# Autodesk Inventor assembly: COTS_ARMA_AR3603_Hinge
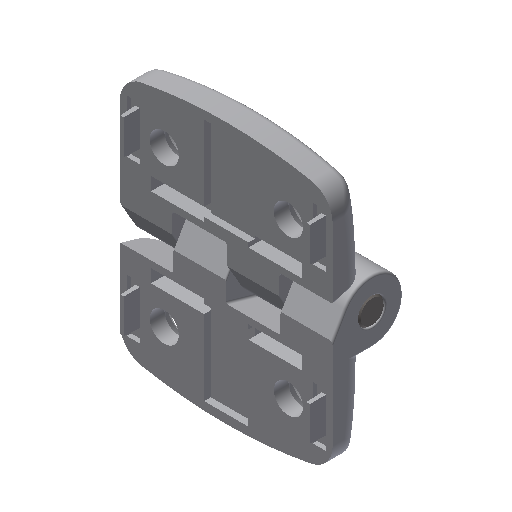
[picture p0: Inventor's stored thumbnail of the model, 512x512]
Saved by Autodesk Inventor 2026.1 (Build 301233000, 233)
## iProperties
Created: 2016-06-24
Part Number: COTS_ARMA_AR3603_Hinge
Material: Ogólny
Document SubType Name: Assembly
Designer: Andrzej
Sending System: Autodesk Inventor 2013
Preprocessor: Autodesk Inventor 2013
Title: \\WIN\Rysunki\Inventor\@System profili aluminiowych\System profili aluminiowych STEP ARMA\AR3603.stp
Author: Konstruktor II
## Documents named in this file (4)
- C:\Users\Andrzej\OneDrive\_DRIVE_SYNCH_FILES\__ BYTECHLAB PROJECTS\MECH - FDM 3D Printer - RAPTOR-360\MCAD\1_REV1\__COTS_PARTS\COTS_ARMA_AR3603_Hinge\COTS_ARMA_AR3603_Hinge.iam
- C:\Users\Andrzej\OneDrive\_DRIVE_SYNCH_FILES\__ BYTECHLAB PROJECTS\MECH - FDM 3D Printer - RAPTOR-360\MCAD\1_REV1\__COTS_PARTS\COTS_ARMA_AR3603_Hinge\AR3603 1.ipt
- C:\Users\Andrzej\OneDrive\_DRIVE_SYNCH_FILES\__ BYTECHLAB PROJECTS\MECH - FDM 3D Printer - RAPTOR-360\MCAD\1_REV1\__COTS_PARTS\COTS_ARMA_AR3603_Hinge\AR3603 2.ipt
- C:\Users\Andrzej\OneDrive\_DRIVE_SYNCH_FILES\__ BYTECHLAB PROJECTS\MECH - FDM 3D Printer - RAPTOR-360\MCAD\1_REV1\__COTS_PARTS\COTS_ARMA_AR3603_Hinge\AR3603 3.ipt
## Components (3 placed, 3 different names)
1. AR3603 1:1 — Styczny:1, Równoległy:1, Zestawiający:1
2. AR3603 2:1 — Styczny:2, Zestawiający:1
3. AR3603 3:1 — Styczny:1, Równoległy:1, Styczny:2
## Relationships (4: Tangent 2, Flush 1, Mate 1)
- Styczny:1 [Tangent]: AR3603 1:1 ↔ AR3603 3:1
- Równoległy:1 [Flush]: AR3603 1:1 ↔ AR3603 3:1
- Styczny:2 [Tangent]: AR3603 2:1 ↔ AR3603 3:1
- Zestawiający:1 [Mate] (0.2 mm): AR3603 1:1 ↔ AR3603 2:1
